# Autodesk Inventor assembly: Washer and bolt combo
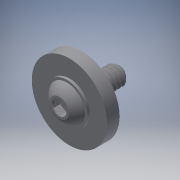
[picture p0: Inventor's stored thumbnail of the model, 180x180]
Saved by Autodesk Inventor 2018 (Build 220112000, 112)
## iProperties
Created: 2020-05-06
Part Number: Washer and bolt combo
Document SubType Name: Assembly
Designer: maste
Author: maste
## Documents named in this file (3)
- C:\Users\maste\OneDrive\Documents\GitHub\2020CAD\Offseason Stuff\swerve but cooler\Part Files\Washer and bolt combo.iam
- C:\Users\maste\OneDrive\Documents\GitHub\2020CAD\Offseason Stuff\swerve but cooler\Part Files\91355A110_FLANGED BUTTON-HEAD SOCKET CAP SCREW.ipt
- C:\Users\maste\OneDrive\Documents\GitHub\2020CAD\Offseason Stuff\swerve but cooler\Part Files\washerino.ipt
## Components (2 placed, 2 different names)
1. 91355A110_FLANGED BUTTON-HEAD SOCKET CAP SCREW:1 — Mate:1, Mate:2, Rotation:1
2. washerino:1 — Mate:1, Mate:2, Rotation:1
## Relationships (3: Mate 2, RelateRotation 1)
- Mate:1: 91355A110_FLANGED BUTTON-HEAD SOCKET CAP SCREW:1 ↔ washerino:1
- Mate:2: 91355A110_FLANGED BUTTON-HEAD SOCKET CAP SCREW:1 ↔ washerino:1
- Rotation:1 [RelateRotation] (1 ul): 91355A110_FLANGED BUTTON-HEAD SOCKET CAP SCREW:1 ↔ washerino:1
